# Autodesk Inventor assembly: Assembled
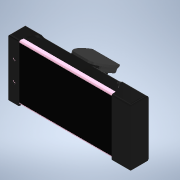
[picture p0: Inventor's stored thumbnail of the model, 180x180]
Saved by Autodesk Inventor 2020 (Build 240168000, 168)
## iProperties
Created: 2020-12-04
Part Number: Assembled
Document SubType Name: Assembly
Designer: Curtis
Author: Curtis
## Documents named in this file (12)
- D:\CAD\leeco-freon\Assembled.iam
- D:\CAD\leeco-freon\heatsink.ipt
- D:\CAD\leeco-freon\leeco.ipt
- D:\CAD\leeco-freon\printed parts\28degree go pro mount.ipt
- D:\CAD\leeco-freon\printed parts\bottomclip.ipt
- D:\CAD\leeco-freon\printed parts\fanduct2.ipt
- D:\CAD\leeco-freon\printed parts\left.ipt
- D:\CAD\leeco-freon\printed parts\right.ipt
- D:\CAD\leeco-freon\printed parts\windshield mount.ipt
- D:\CAD\leeco-freon\noctua fan\NF-A4x10_Noctua_40mm.iam
- D:\CAD\leeco-freon\eonPCB.ipt
- D:\CAD\leeco-freon\printed parts\eonPCBholder.ipt
## Components (11 placed, 11 different names)
1. heatsink:1 — Mate:6, Mate:7, Flush:3
2. leeco:1 — Mate:1, Mate:3, Mate:4, Flush:2, Mate:6, Flush:3, Mate:8, Mate:21, Mate:22, Mate:23
3. 28degree go pro mount:1 — Mate:14, Mate:15, Mate:18, Mate:19, Mate:20
4. bottomclip:1 — Mate:16, Mate:17
5. fanduct2:1 — Mate:8, Mate:9, Mate:10, Mate:12, Mate:13
6. left:1 — Mate:4, Flush:1, Mate:5, Mate:7, Mate:14, Mate:16
7. right:1 — Mate:1, Mate:3, Flush:1, Mate:5, Flush:2, Mate:9, Mate:10, Mate:11, Mate:15, Mate:17, Mate:24, Mate:25
8. windshield mount:1 — Mate:18, Mate:19, Mate:20
9. NF-A4x10_Noctua_40mm:1 [sub-assembly] — Mate:11, Mate:12, Mate:13
10. eonPCB:1 — Mate:21, Mate:22, Mate:23
11. eonPCBholder:1 — Mate:24, Mate:25
## Relationships (27: Mate 24, Flush 3)
- Mate:1: leeco:1 ↔ right:1
- Mate:3: leeco:1 ↔ right:1
- Mate:4: leeco:1 ↔ left:1
- Flush:1: left:1 ↔ right:1
- Mate:5: left:1 ↔ right:1
- Flush:2: leeco:1 ↔ right:1
- Mate:6: heatsink:1 ↔ leeco:1
- Mate:7: heatsink:1 ↔ left:1
- Flush:3 (7 mm): heatsink:1 ↔ leeco:1
- Mate:8: leeco:1 ↔ fanduct2:1
- Mate:9: fanduct2:1 ↔ right:1
- Mate:10: fanduct2:1 ↔ right:1
- Mate:11: right:1 ↔ NF-A4x10_Noctua_40mm:1
- Mate:12: fanduct2:1 ↔ NF-A4x10_Noctua_40mm:1
- Mate:13: fanduct2:1 ↔ NF-A4x10_Noctua_40mm:1
- Mate:14: 28degree go pro mount:1 ↔ left:1
- Mate:15: 28degree go pro mount:1 ↔ right:1
- Mate:16: bottomclip:1 ↔ left:1
- Mate:17: bottomclip:1 ↔ right:1
- Mate:18: 28degree go pro mount:1 ↔ windshield mount:1
- Mate:19 (0.1 mm): 28degree go pro mount:1 ↔ windshield mount:1
- Mate:20: 28degree go pro mount:1 ↔ windshield mount:1
- Mate:21: leeco:1 ↔ eonPCB:1
- Mate:22: leeco:1 ↔ eonPCB:1
- Mate:23: leeco:1 ↔ eonPCB:1
- Mate:24: right:1 ↔ eonPCBholder:1
- Mate:25: right:1 ↔ eonPCBholder:1
